# Autodesk Inventor assembly: RadLWL
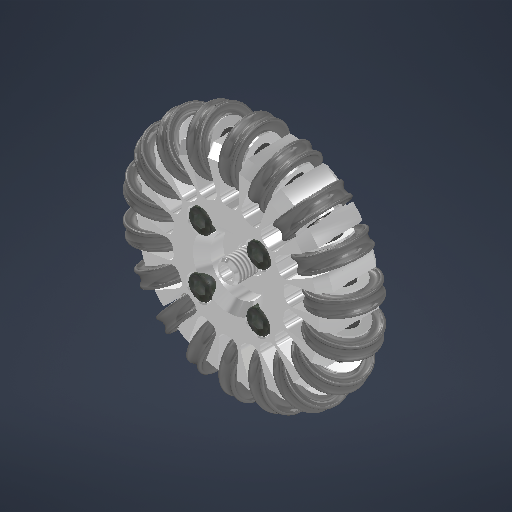
[picture p0: Inventor's stored thumbnail of the model, 512x512]
Saved by Autodesk Inventor 2026.1 (Build 301233020, 233B)
## iProperties
Created: 2025-03-24
Part Number: RadLWL
Document SubType Name: Assembly
Designer: Faabs
Mass: 29.0877 g
Surface Area: 292.171 cm^2
Volume: 19.2019 cm^3
Density: 1.51483 g/cm^3
Author: Faabs
## Documents named in this file (6)
- C:\Users\Bahaa\Nextcloud2\CAD\25-26\V2\RadLWL\RadLWL.iam
- C:\Users\Bahaa\Nextcloud2\CAD\25-26\V2\RadLWL\Radkasten.ipt
- C:\Users\Bahaa\Nextcloud2\CAD\25-26\V2\RadLWL\Rolle\UBG-Rolle.iam
- C:\Users\Bahaa\Nextcloud2\CAD\25-26\V2\RadLWL\Raddeckel.ipt
- C:\Users\Bahaa\Nextcloud2\CAD\25-26\V2\RadLWL\DIN 912 - M3 x 0,5 x 6 x 4,75.ipt
- C:\Users\Bahaa\Nextcloud2\CAD\25-26\V2\RadLWL\Radadapter.ipt
## Components (25 placed, 5 different names)
1. Radkasten:1 — Flush:1, Flush:2, Flush:3, Mate:1, Mate:2, Mate:4, Mate:5, Mate:7, Mate:8, Mate:15, Mate:16, Angle:1
2. Raddeckel:1 — Mate:4, Mate:5, Mate:8, Insert:1, Insert:2, Insert:3, Insert:4
3. Radadapter:1 — Mate:15, Mate:16, Angle:1
4. DIN 912 - ersetzt durch DIN EN ISO 4762 M3 x 6:4 — Insert:1
5. DIN 912 - ersetzt durch DIN EN ISO 4762 M3 x 6:3 — Insert:3
6. DIN 912 - ersetzt durch DIN EN ISO 4762 M3 x 6:2 — Insert:4
7. DIN 912 - ersetzt durch DIN EN ISO 4762 M3 x 6:1 — Insert:2
8. UBG-Rolle:1 [sub-assembly] — Mate:1, Mate:2, Mate:7
9. UBG-Rolle:2 [sub-assembly]
10. UBG-Rolle:3 [sub-assembly]
11. UBG-Rolle:4 [sub-assembly]
12. UBG-Rolle:5 [sub-assembly]
13. UBG-Rolle:6 [sub-assembly]
14. UBG-Rolle:7 [sub-assembly]
15. UBG-Rolle:8 [sub-assembly]
16. UBG-Rolle:9 [sub-assembly]
17. UBG-Rolle:10 [sub-assembly]
18. UBG-Rolle:11 [sub-assembly]
19. UBG-Rolle:12 [sub-assembly]
20. UBG-Rolle:13 [sub-assembly]
21. UBG-Rolle:14 [sub-assembly]
22. UBG-Rolle:15 [sub-assembly]
23. UBG-Rolle:16 [sub-assembly]
24. UBG-Rolle:17 [sub-assembly]
25. UBG-Rolle:18 [sub-assembly]
## Component patterns: (18 elements, first: UBG-Rolle:1)
## Relationships (16: Mate 8, Insert 4, Flush 3, Angle 1)
- Flush:1: Radkasten:1
- Flush:2: Radkasten:1
- Flush:3: Radkasten:1
- Mate:1: Radkasten:1 ↔ UBG-Rolle:1
- Mate:2 (0.2 mm): Radkasten:1 ↔ UBG-Rolle:1
- Mate:4: Radkasten:1 ↔ Raddeckel:1
- Mate:5: Radkasten:1 ↔ Raddeckel:1
- Mate:7 (7 mm): Radkasten:1 ↔ UBG-Rolle:1
- Mate:8: Radkasten:1 ↔ Raddeckel:1
- Insert:1: Raddeckel:1 ↔ DIN 912 - ersetzt durch DIN EN ISO 4762 M3 x 6:4
- Insert:2: Raddeckel:1 ↔ DIN 912 - ersetzt durch DIN EN ISO 4762 M3 x 6:1
- Insert:3: Raddeckel:1 ↔ DIN 912 - ersetzt durch DIN EN ISO 4762 M3 x 6:3
- Insert:4: Raddeckel:1 ↔ DIN 912 - ersetzt durch DIN EN ISO 4762 M3 x 6:2
- Mate:15: Radkasten:1 ↔ Radadapter:1
- Mate:16: Radkasten:1 ↔ Radadapter:1
- Angle:1 (0 deg): Radkasten:1 ↔ Radadapter:1
